# Autodesk Inventor assembly: Chassis
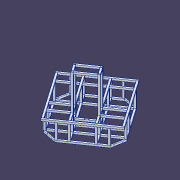
[picture p0: Inventor's stored thumbnail of the model, 180x180]
Saved by Autodesk Inventor 2017 SP1 (Build 210196100, 196)
## iProperties
Created: 2017-06-13
Part Number: Chassis
Document SubType Name: Assembly
Designer: zallen
Mass: 2624.68 g
Surface Area: 12822.9 cm^2
Volume: 1698.76 cm^3
Density: 1.54505 g/cm^3
Author: zallen
## Documents named in this file (14)
- C:\Users\Zach\Documents\GitHub\tr1\src\Base\Chassis\Chassis.iam
- C:\Users\Zach\Documents\GitHub\tr1\src\Base\Chassis\C001.ipt
- C:\Users\Zach\Documents\GitHub\tr1\src\Base\Chassis\C002.ipt
- C:\Users\Zach\Documents\GitHub\tr1\src\Base\Chassis\C003.ipt
- C:\Users\Zach\Documents\GitHub\tr1\src\Base\Chassis\C006.ipt
- C:\Users\Zach\Documents\GitHub\tr1\src\Base\Chassis\C007.ipt
- C:\Users\Zach\Documents\GitHub\tr1\src\Base\Chassis\C008.ipt
- C:\Users\Zach\Documents\GitHub\tr1\src\Base\Chassis\C010.ipt
- C:\Users\Zach\Documents\GitHub\tr1\src\Base\Chassis\C009.ipt
- C:\Users\Zach\Documents\GitHub\tr1\src\Base\Chassis\C011.ipt
- C:\Users\Zach\Documents\GitHub\tr1\src\Base\Chassis\C012.ipt
- C:\Users\Zach\Documents\GitHub\tr1\src\Base\Chassis\C013.ipt
- C:\Users\Zach\Documents\GitHub\tr1\src\Base\Chassis\C014.ipt
- C:\Users\Zach\Documents\GitHub\tr1\src\Base\Chassis\C015.ipt
## Components (67 placed, 13 different names)
1. C001:1 — Mate:2, Mate:3, Mate:10, Mate:11, Mate:67, Mate:69, Mate:70, Flush:187, Mate:187, Mate:188, Mate:201, Mate:202
2. C001:2 — Mate:4, Mate:5, Mate:12, Mate:13, Mate:64, Mate:65, Mate:189, Mate:190
3. C002:1 — Mate:2, Mate:3, Mate:6, Mate:7
4. C002:2 — Mate:4, Mate:5, Mate:8, Mate:9, Mate:66, Mate:76
5. C003:1 — Mate:6, Mate:7, Mate:8, Mate:9, Mate:75, Mate:77, Mate:78, Mate:135, Mate:143, Flush:199, Mate:198
6. C002:3 — Mate:10, Mate:11, Mate:68, Mate:74
7. C002:4 — Mate:12, Mate:13, Mate:14, Mate:17, Mate:60, Mate:61, Mate:62, Mate:63
8. C003:2 — Mate:14, Mate:17, Mate:60, Mate:61, Mate:62, Mate:71, Mate:72, Mate:73, Mate:130, Mate:165, Flush:195, Mate:197, Mate:234
9. C006:1 — Mate:63, Mate:64, Flush:191
10. C006:2 — Mate:65, Mate:66, Mate:87, Mate:88, Flush:192
11. C006:3 — Mate:67, Mate:68
12. C006:4 — Mate:69, Mate:70, Mate:89, Mate:90
13. C006:5 — Mate:71, Mate:72, Mate:221
14. C006:6 — Mate:73, Mate:74, Flush:196
15. C006:7 — Mate:75, Mate:76, Flush:216
16. C006:8 — Mate:77, Mate:78, Mate:208
17. C007:1 — Mate:87, Mate:88, Flush:19, Flush:21, Mate:179, Mate:213, Mate:214, Mate:224, Mate:225
18. C007:2 — Mate:89, Mate:90, Flush:221, Flush:223, Mate:217, Mate:218, Mate:233
19. C008:3 — Mate:109, Mate:110, Mate:113, Mate:115, Mate:124, Mate:131, Mate:132, Mate:176, Flush:11, Flush:13, Flush:14, Mate:178, Flush:22, Mate:181, Flush:194, Mate:205
20. C008:4 — Mate:111, Mate:112, Mate:114, Mate:116, Mate:127, Mate:133, Mate:134, Flush:1, Flush:4, Mate:170, Mate:171, Mate:173, Flush:24, Flush:25, Mate:180, Mate:183, Flush:193, Flush:225, Mate:203
21. C010:1 — Mate:109, Mate:110, Mate:111, Mate:112
22. C010:2 — Mate:113, Mate:114, Mate:115, Mate:116, Flush:18
23. C009:1 — Mate:124, Mate:223
24. C009:2 — Mate:127, Mate:216
25. C009:3 — Mate:130, Mate:131, Mate:132, Mate:226
26. C009:4 — Mate:133, Mate:134, Mate:135, Flush:6
27. C009:5 — Mate:144, Flush:5, Flush:215, Mate:215
28. C009:6 — Mate:143, Mate:145, Mate:146
29. C008:5 — Mate:144, Mate:145, Mate:146, Mate:153, Mate:154, Mate:172, Mate:174, Mate:175, Flush:26
30. C010:3 — Mate:153, Mate:154, Mate:155, Mate:156, Mate:163
31. C008:6 — Mate:155, Mate:156, Mate:164, Mate:166, Mate:168, Mate:169, Flush:9, Flush:12, Mate:177, Flush:226, Mate:207, Mate:228
32. C009:7 — Mate:163, Mate:164, Mate:165, Flush:16, Flush:190
33. C009:8 — Mate:166, Flush:17, Flush:213, Mate:219, Flush:232
34. C010:4 — Mate:168, Mate:169, Flush:8, Mate:175, Flush:10
35. C011:1 — Flush:13, Flush:16, Mate:178, Flush:189, Flush:230
36. C011:2 — Flush:14, Mate:177, Flush:17, Flush:231
37. C011:4 — Flush:8, Flush:9, Mate:176, Flush:11, Flush:12
38. C011:5 — Flush:4, Flush:5, Mate:173
39. C011:6 — Flush:1, Mate:170, Mate:171, Mate:172, Flush:10
40. C011:7 — Flush:6, Mate:174, Flush:26, Flush:188, Mate:204
41. C012:1 — Flush:18, Flush:25, Mate:183
42. C012:2 — Flush:19, Flush:24, Mate:179, Mate:180
43. C012:3 — Flush:21, Flush:22, Mate:181
44. C013:1 — Flush:187, Mate:187, Flush:188, Mate:192, Mate:193, Flush:202, Mate:195
45. C013:2 — Flush:189, Flush:190, Mate:188, Mate:191, Flush:198, Flush:203, Mate:194
46. C006:9 — Flush:191, Mate:190, Flush:193
47. C006:10 — Flush:192, Mate:189, Flush:194, Mate:227
48. C010:5 — Flush:197, Flush:198, Mate:192, Flush:200, Flush:201
49. C009:9 — Flush:199, Flush:200, Mate:193
50. C009:10 — Flush:195, Mate:191, Flush:196, Flush:197, Flush:204
51. C006:11 — Flush:203, Flush:204, Mate:194, Mate:199
52. C006:12 — Flush:201, Flush:202, Mate:195, Flush:212
53. C010:6 — Flush:212, Flush:217, Flush:219, Mate:230, Mate:231
54. C006:13 — Flush:213, Mate:197, Mate:211, Mate:220
55. C006:14 — Flush:215, Flush:216, Mate:198
56. C009:11 — Flush:219, Mate:199, Mate:212, Mate:222, Mate:229
57. C009:12 — Flush:217, Mate:210, Mate:232
58. C006:15 — Flush:221, Mate:201, Flush:233
59. C006:16 — Flush:223, Mate:202, Flush:234
60. C011:8 — Flush:225, Mate:203, Mate:204, Flush:227, Flush:229, Mate:206
61. C011:9 — Flush:226, Mate:205, Flush:227
62. C014:1 — Flush:229, Mate:206, Mate:207
63. C015:1 — Mate:211, Mate:212, Mate:218, Mate:219, Mate:220, Mate:221, Mate:222, Mate:223, Mate:224, Mate:225
64. C015:2 — Mate:208, Mate:210, Mate:213, Mate:214, Mate:215, Mate:216, Mate:217
65. C012:6 — Flush:230, Mate:226, Mate:227
66. C013:3 — Mate:231, Mate:232, Mate:233, Flush:233
67. C013:4 — Mate:228, Flush:231, Flush:232, Mate:229, Mate:230, Flush:234
## Relationships (180: Mate 125, Flush 55)
- Mate:2: C001:1 ↔ C002:1
- Mate:3: C001:1 ↔ C002:1
- Mate:4: C001:2 ↔ C002:2
- Mate:5: C001:2 ↔ C002:2
- Mate:6: C002:1 ↔ C003:1
- Mate:7: C002:1 ↔ C003:1
- Mate:8: C002:2 ↔ C003:1
- Mate:9: C002:2 ↔ C003:1
- Mate:10: C001:1 ↔ C002:3
- Mate:11: C001:1 ↔ C002:3
- Mate:12: C001:2 ↔ C002:4
- Mate:13: C001:2 ↔ C002:4
- Mate:14: C002:4 ↔ C003:2
- Mate:17: C002:4 ↔ C003:2
- Mate:60: C002:4 ↔ C003:2
- Mate:61: C002:4 ↔ C003:2
- Mate:62: C002:4 ↔ C003:2
- Mate:63: C002:4 ↔ C006:1
- Mate:64: C001:2 ↔ C006:1
- Mate:65: C001:2 ↔ C006:2
- Mate:66: C002:2 ↔ C006:2
- Mate:67: C001:1 ↔ C006:3
- Mate:68: C002:3 ↔ C006:3
- Mate:69: C001:1 ↔ C006:4
- Mate:70: C001:1 ↔ C006:4
- Mate:71: C003:2 ↔ C006:5
- Mate:72: C003:2 ↔ C006:5
- Mate:73: C003:2 ↔ C006:6
- Mate:74: C002:3 ↔ C006:6
- Mate:75: C003:1 ↔ C006:7
- Mate:76: C002:2 ↔ C006:7
- Mate:77: C003:1 ↔ C006:8
- Mate:78: C003:1 ↔ C006:8
- Mate:87: C006:2 ↔ C007:1
- Mate:88: C006:2 ↔ C007:1
- Mate:89: C006:4 ↔ C007:2
- Mate:90: C006:4 ↔ C007:2
- Mate:109: C008:3 ↔ C010:1
- Mate:110: C008:3 ↔ C010:1
- Mate:111: C008:4 ↔ C010:1
- Mate:112: C008:4 ↔ C010:1
- Mate:113: C008:3 ↔ C010:2
- Mate:114: C008:4 ↔ C010:2
- Mate:115: C008:3 ↔ C010:2
- Mate:116: C008:4 ↔ C010:2
- Mate:124: C008:3 ↔ C009:1
- Mate:127: C008:4 ↔ C009:2
- Mate:130: C003:2 ↔ C009:3
- Mate:131: C008:3 ↔ C009:3
- Mate:132: C008:3 ↔ C009:3
- Mate:133: C008:4 ↔ C009:4
- Mate:134: C008:4 ↔ C009:4
- Mate:135: C003:1 ↔ C009:4
- Mate:143: C003:1 ↔ C009:6
- Mate:144: C009:5 ↔ C008:5
- Mate:145: C009:6 ↔ C008:5
- Mate:146: C009:6 ↔ C008:5
- Mate:153: C008:5 ↔ C010:3
- Mate:154: C008:5 ↔ C010:3
- Mate:155: C010:3 ↔ C008:6
- Mate:156: C010:3 ↔ C008:6
- Mate:163: C010:3 ↔ C009:7
- Mate:164: C008:6 ↔ C009:7
- Mate:165: C003:2 ↔ C009:7
- Mate:166: C008:6 ↔ C009:8
- Mate:168: C008:6 ↔ C010:4
- Mate:169: C008:6 ↔ C010:4
- Flush:1: C008:4 ↔ C011:6
- Flush:4: C008:4 ↔ C011:5
- Flush:5: C009:5 ↔ C011:5
- Mate:170: C008:4 ↔ C011:6
- Mate:171: C008:4 ↔ C011:6
- Mate:172: C008:5 ↔ C011:6
- Mate:173: C008:4 ↔ C011:5
- Flush:6: C009:4 ↔ C011:7
- Mate:174: C008:5 ↔ C011:7
- Flush:8: C010:4 ↔ C011:4
- Flush:9: C008:6 ↔ C011:4
- Mate:175: C008:5 ↔ C010:4
- Flush:10: C010:4 ↔ C011:6
- Mate:176: C008:3 ↔ C011:4
- Flush:11: C008:3 ↔ C011:4
- Flush:12: C008:6 ↔ C011:4
- Flush:13: C008:3 ↔ C011:1
- Flush:14: C008:3 ↔ C011:2
- Mate:177: C008:6 ↔ C011:2
- Flush:16: C009:7 ↔ C011:1
- Mate:178: C008:3 ↔ C011:1
- Flush:17: C009:8 ↔ C011:2
- Flush:18: C010:2 ↔ C012:1
- Flush:19: C007:1 ↔ C012:2
- Flush:21: C007:1 ↔ C012:3
- Flush:22: C008:3 ↔ C012:3
- Flush:24: C008:4 ↔ C012:2
- Flush:25: C008:4 ↔ C012:1
- Mate:179: C007:1 ↔ C012:2
- Mate:180: C008:4 ↔ C012:2
- Mate:181: C008:3 ↔ C012:3
- Mate:183: C008:4 ↔ C012:1
- Flush:26: C008:5 ↔ C011:7
- Flush:187: C001:1 ↔ C013:1
- Mate:187: C001:1 ↔ C013:1
- Flush:188: C011:7 ↔ C013:1
- Flush:189: C011:1 ↔ C013:2
- Flush:190: C009:7 ↔ C013:2
- Mate:188: C001:1 ↔ C013:2
- Flush:191: C006:1 ↔ C006:9
- Flush:192: C006:2 ↔ C006:10
- Mate:189: C001:2 ↔ C006:10
- Mate:190: C001:2 ↔ C006:9
- Flush:193: C008:4 ↔ C006:9
- Flush:194: C008:3 ↔ C006:10
- Flush:195: C003:2 ↔ C009:10
- Mate:191: C013:2 ↔ C009:10
- Flush:196: C006:6 ↔ C009:10
- Flush:197: C010:5 ↔ C009:10
- Flush:198: C013:2 ↔ C010:5
- Mate:192: C013:1 ↔ C010:5
- Flush:199: C003:1 ↔ C009:9
- Flush:200: C010:5 ↔ C009:9
- Mate:193: C013:1 ↔ C009:9
- Flush:201: C010:5 ↔ C006:12
- Flush:202: C013:1 ↔ C006:12
- Flush:203: C013:2 ↔ C006:11
- Flush:204: C009:10 ↔ C006:11
- Mate:194: C013:2 ↔ C006:11
- Mate:195: C013:1 ↔ C006:12
- Flush:212: C006:12 ↔ C010:6
- Flush:213: C009:8 ↔ C006:13
- Mate:197: C003:2 ↔ C006:13
- Flush:215: C009:5 ↔ C006:14
- Flush:216: C006:7 ↔ C006:14
- Mate:198: C003:1 ↔ C006:14
- Flush:217: C010:6 ↔ C009:12
- Flush:219: C010:6 ↔ C009:11
- Mate:199: C006:11 ↔ C009:11
- Flush:221: C007:2 ↔ C006:15
- Flush:223: C007:2 ↔ C006:16
- Mate:201: C001:1 ↔ C006:15
- Mate:202: C001:1 ↔ C006:16
- Flush:225: C008:4 ↔ C011:8
- Mate:203: C008:4 ↔ C011:8
- Mate:204 (66 mm): C011:7 ↔ C011:8
- Flush:226: C008:6 ↔ C011:9
- Mate:205: C008:3 ↔ C011:9
- Flush:227: C011:8 ↔ C011:9
- Flush:229: C011:8 ↔ C014:1
- Mate:206: C011:8 ↔ C014:1
- Mate:207 (28 mm): C008:6 ↔ C014:1
- Mate:208: C006:8 ↔ C015:2
- Mate:210: C009:12 ↔ C015:2
- Mate:211: C006:13 ↔ C015:1
- Mate:212: C009:11 ↔ C015:1
- Mate:213: C007:1 ↔ C015:2
- Mate:214: C007:1 ↔ C015:2
- Mate:215: C009:5 ↔ C015:2
- Mate:216: C009:2 ↔ C015:2
- Mate:217: C007:2 ↔ C015:2
- Mate:218: C007:2 ↔ C015:1
- Mate:219: C009:8 ↔ C015:1
- Mate:220: C006:13 ↔ C015:1
- Mate:221: C006:5 ↔ C015:1
- Mate:222: C009:11 ↔ C015:1
- Mate:223: C009:1 ↔ C015:1
- Mate:224: C007:1 ↔ C015:1
- Mate:225: C007:1 ↔ C015:1
- Flush:230: C011:1 ↔ C012:6
- Mate:226: C009:3 ↔ C012:6
- Mate:227: C006:10 ↔ C012:6
- Mate:228: C008:6 ↔ C013:4
- Flush:231: C011:2 ↔ C013:4
- Flush:232: C009:8 ↔ C013:4
- Mate:229: C009:11 ↔ C013:4
- Mate:230: C010:6 ↔ C013:4
- Mate:231: C010:6 ↔ C013:3
- Mate:232: C009:12 ↔ C013:3
- Mate:233: C007:2 ↔ C013:3
- Mate:234: C003:2
- Flush:233: C006:15 ↔ C013:3
- Flush:234: C006:16 ↔ C013:4
